# Autodesk Inventor assembly: third_floor
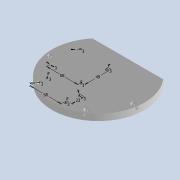
[picture p0: Inventor's stored thumbnail of the model, 180x180]
Saved by Autodesk Inventor 2020.4 (Build 244396000, 396)
## iProperties
Created: 2021-05-06
Part Number: third_floor
Document SubType Name: Assembly
Designer: Acer
Author: Acer
## Documents named in this file (4)
- G:\Meu Drive\RobôCIn\Mecânica\SSL\2021\vRoboCup2021\third_floor\third_floor.iam
- G:\Meu Drive\RobôCIn\Mecânica\SSL\2021\vRoboCup2021\third_floor\plate_third_floor.ipt
- G:\Meu Drive\RobôCIn\Mecânica\SSL\2021\vRoboCup2021\third_floor\raspberry-pi-4-model-b-1.snapshot.3\Raspberry Pi 4 Model B.iam
- G:\Meu Drive\RobôCIn\Mecânica\SSL\2021\vRoboCup2021\third_floor\coral-usb-accelerator-1.snapshot.3 (1)\Coral USB Accelerator v1.ipt
## Components (3 placed, 3 different names)
1. plate_third_floor:1 — Mate:1, Mate:2, Mate:3, Mate:4, Mate:5, Mate:6
2. Raspberry Pi 4 Model B:1 [sub-assembly] — Mate:1, Mate:2, Mate:3
3. Coral USB Accelerator v1:1 — Mate:4, Mate:5, Mate:6
## Relationships (6: Mate 6)
- Mate:1: plate_third_floor:1 ↔ Raspberry Pi 4 Model B:1
- Mate:2: plate_third_floor:1 ↔ Raspberry Pi 4 Model B:1
- Mate:3: plate_third_floor:1 ↔ Raspberry Pi 4 Model B:1
- Mate:4: plate_third_floor:1 ↔ Coral USB Accelerator v1:1
- Mate:5: plate_third_floor:1 ↔ Coral USB Accelerator v1:1
- Mate:6: plate_third_floor:1 ↔ Coral USB Accelerator v1:1
